# Autodesk Inventor assembly: SparkFun USB Type A Female Breakout
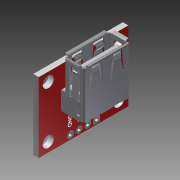
[picture p0: Inventor's stored thumbnail of the model, 180x180]
Saved by Autodesk Inventor 2013 SP2 (Build 170200200, 200)
## iProperties
Created: 2018-05-07
Part Number: SparkFun USB Type A Female Breakout
Document SubType Name: Assembly
Designer: PCC
Author: PCC
## Documents named in this file (3)
- D:\Dokumenty\Projekty\Inventor projekty\TimeLapse\TimeLapse HAKA 01\Importované komponenty\Konektory\USB\SparkFun USB Type A Female Breakout\SparkFun USB Type A Female Breakout.iam
- D:\Dokumenty\Projekty\Inventor projekty\TimeLapse\TimeLapse HAKA 01\Importované komponenty\Konektory\USB\SparkFun USB Type A Female Breakout\SparkFun USB Type A Female Breakout - doska.ipt
- D:\Dokumenty\Projekty\Inventor projekty\TimeLapse\TimeLapse HAKA 01\Importované komponenty\Konektory\USB\SparkFun USB Type A Female Breakout\femaleThruHoleUSB.ipt
## Components (2 placed, 2 different names)
1. SparkFun USB Type A Female Breakout - doska:1 — Proti sobě:1, Stejný směr:1, Proti sobě:2
2. femaleThruHoleUSB:1 — Proti sobě:1, Stejný směr:1, Proti sobě:2
## Relationships (3: Mate 2, Flush 1)
- Proti sobě:1 [Mate]: SparkFun USB Type A Female Breakout - doska:1 ↔ femaleThruHoleUSB:1
- Stejný směr:1 [Flush] (-6.445 mm): SparkFun USB Type A Female Breakout - doska:1 ↔ femaleThruHoleUSB:1
- Proti sobě:2 [Mate] (-23 mm): SparkFun USB Type A Female Breakout - doska:1 ↔ femaleThruHoleUSB:1
